# Autodesk Inventor assembly: DoorAssembly
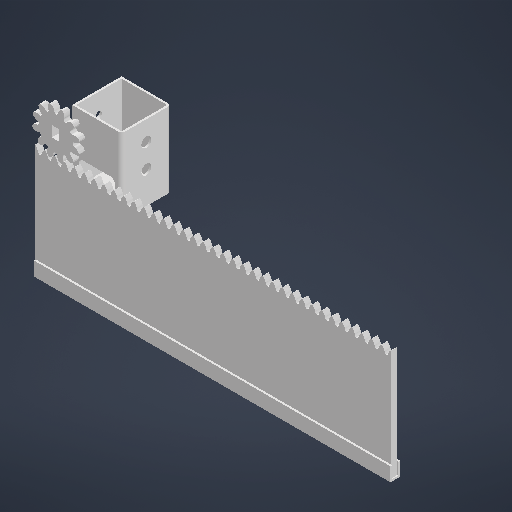
[picture p0: Inventor's stored thumbnail of the model, 512x512]
Saved by Autodesk Inventor 2026.1 (Build 301233000, 233)
## iProperties
Created: 2026-02-26
Part Number: DoorAssembly
Document SubType Name: Assembly
Designer: ba2032
Author: ba2032
## Documents named in this file (5)
- C:\Users\ba2032\Documents\DoorAssembly.iam
- H:\CAD Project\DoorPinion.ipt
- H:\CAD Project\Door.ipt
- H:\CAD Project\DoorRail.ipt
- H:\CAD Project\MotorHolder.ipt
## Components (4 placed, 4 different names)
1. DoorPinion:1 — Mate:1, Flush:1, Mate:2
2. Door:1 — Flush:2, Mate:2, Flush:3, Slider:1, Flush:4
3. DoorRail:1 — Slider:1, Flush:4, Mate:3
4. MotorHolder:1
## Relationships (8: Flush 4, Mate 3, TranslationJoint 1)
- Mate:1: DoorPinion:1
- Flush:1: DoorPinion:1
- Flush:2: Door:1
- Mate:2 (254 mm): DoorPinion:1 ↔ Door:1
- Flush:3 (254 mm): Door:1
- Slider:1 [TranslationJoint]: Door:1 ↔ DoorRail:1
- Flush:4 (-25.4 mm): Door:1 ↔ DoorRail:1
- Mate:3 (-254 mm): DoorRail:1
